# Autodesk Inventor assembly: Servo mount + servo
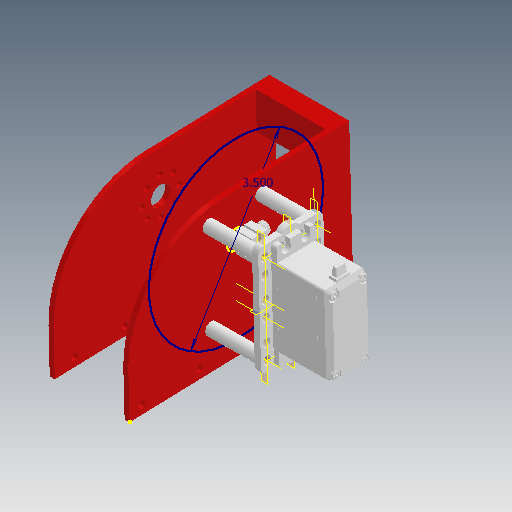
[picture p0: Inventor's stored thumbnail of the model, 512x512]
Saved by Autodesk Inventor 2020 (Build 240168000, 168)
## iProperties
Created: 2020-01-01
Part Number: Servo mount + servo
Document SubType Name: Assembly
Designer: ball
Author: ball
## Documents named in this file (3)
- C:\FTC\FTC8863CAD\2019 Robot\Delivery\extension arm\Servo mount + servo.iam
- C:\FTC\FTC8863CAD\2019 Robot\Delivery\extension arm\whole servo mount.ipt
- C:\FTC\FTC8863CAD\2019 Robot\Delivery\extension arm\servo.iam
## Components (2 placed, 2 different names)
1. whole servo mount:1
2. servo:1 [sub-assembly]
## Relationships (2: Mate 2)
- [Mate]: whole servo mount:1 ↔ servo:1
- [Mate]: whole servo mount:1 ↔ servo:1
